# Autodesk Inventor assembly: 2K8 FEET long
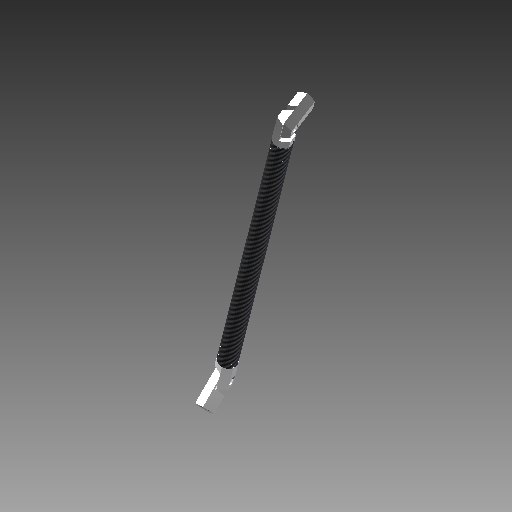
[picture p0: Inventor's stored thumbnail of the model, 512x512]
Saved by Autodesk Inventor 2018 (Build 220112000, 112)
## iProperties
Created: 2018-12-06
Part Number: 2K8 FEET long
Document SubType Name: Assembly
Designer: freyja
Author: freyja
## Documents named in this file (4)
- C:\Users\freyja\Documents\Cryostat\CAD\2K8 FEET long.iam
- C:\Users\freyja\Documents\Cryostat\CAD\feet type 3 part 1 hexagon stock 10-32 hole.ipt
- C:\Users\freyja\Documents\Cryostat\CAD\feet type 3 part 2 hex stock 10-32.ipt
- C:\Users\freyja\Documents\Cryostat\CAD\feet type 3 part 3 2k8 length.ipt
## Components (5 placed, 3 different names)
1. feet type 3 part 1 hexagon stock 10-32 hole:1 — Rotational:2
2. feet type 3 part 1 hexagon stock 10-32 hole:2 — Rotational:1
3. feet type 3 part 2 hex stock 10-32:1 — Mate:3, Mate:4, Rotational:2, Mate:5
4. feet type 3 part 2 hex stock 10-32:2 — Mate:1, Rotational:1, Mate:5, Mate:6
5. feet type 3 part 3 2k8 length:1 — Mate:1, Mate:3, Mate:4, Mate:6
## Relationships (7: Mate 5, RevoluteJoint 2)
- Mate:1: feet type 3 part 2 hex stock 10-32:2 ↔ feet type 3 part 3 2k8 length:1
- Mate:3: feet type 3 part 2 hex stock 10-32:1 ↔ feet type 3 part 3 2k8 length:1
- Mate:4: feet type 3 part 2 hex stock 10-32:1 ↔ feet type 3 part 3 2k8 length:1
- Rotational:1 [RevoluteJoint]: feet type 3 part 1 hexagon stock 10-32 hole:2 ↔ feet type 3 part 2 hex stock 10-32:2
- Rotational:2 [RevoluteJoint]: feet type 3 part 1 hexagon stock 10-32 hole:1 ↔ feet type 3 part 2 hex stock 10-32:1
- Mate:5: feet type 3 part 2 hex stock 10-32:1 ↔ feet type 3 part 2 hex stock 10-32:2
- Mate:6: feet type 3 part 2 hex stock 10-32:2 ↔ feet type 3 part 3 2k8 length:1
